# Autodesk Inventor assembly: ChassisBase
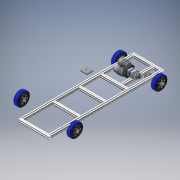
[picture p0: Inventor's stored thumbnail of the model, 180x180]
Saved by Autodesk Inventor 2018 (Build 220112000, 112)
## iProperties
Created: 2017-09-03
Part Number: ChassisBase
Document SubType Name: Assembly
Designer: snipe
Author: snipe
## Documents named in this file (12)
- E:\50000skater\Assets\ChassisBase.iam
- E:\50000skater\Assets\Resources\Profile_Len_860mm.ipt
- E:\50000skater\Assets\Resources\Profile_Len_200mm.ipt
- E:\50000skater\Assets\Resources\Profile_Len_160mm.ipt
- E:\50000skater\Assets\VPlan775dualinput.iam
- E:\50000skater\Assets\24tPulley15mm.ipt
- E:\50000skater\Assets\ShaftCollar.ipt
- E:\50000skater\Assets\PlactionWheelwithHub.iam
- E:\50000skater\Assets\PlactionWheelNoHub.iam
- E:\50000skater\Assets\THex240mm.ipt
- E:\50000skater\Assets\BearingBlock.ipt
- E:\50000skater\Assets\FlangedThunderHexBearing.ipt
## Components (21 placed, 11 different names)
1. Profile_Len_200mm:1 — Mate:1, Mate:2, Mate:3, Flush:1, Flush:2, Mate:4, Flush:3, Flush:4, Mate:10, Mate:11, Mate:13, Flush:10, Mate:23, Flush:12
2. Profile_Len_860mm:1 — Mate:3, Flush:1, Flush:2, Mate:5, Flush:5, Flush:6, Mate:7, Mate:8, Mate:9, Flush:7, Flush:8, Flush:9, Mate:30
3. Profile_Len_860mm:2 — Mate:4, Flush:3, Flush:4, Mate:16, Mate:31
4. Profile_Len_200mm:2 — Mate:5, Flush:5, Flush:6
5. Profile_Len_160mm:1 — Mate:7, Flush:9, Mate:11
6. Profile_Len_160mm:2 — Mate:8, Flush:8, Mate:10
7. Profile_Len_160mm:3 — Mate:9, Flush:7, Mate:14
8. VPlan775dualinput:1 [sub-assembly] — Flush:11, Mate:15, Mate:16, Mate:17, Mate:18, Mate:19, Mate:20, Mate:21
9. Profile_Len_200mm:3 — Mate:13, Flush:10, Mate:14, Flush:11, Mate:15
10. 24tPulley15mm:1 — Mate:17, Mate:18, Mate:19, Mate:22, Flush:13
11. ShaftCollar:1 — Mate:20, Mate:21, Mate:22
12. PlactionWheelwithHub:1 [sub-assembly] — Mate:28, Mate:29, Mate:30, Mate:35
13. PlactionWheelwithHub:2 [sub-assembly] — Mate:26, Mate:27, Mate:31, Mate:32
14. PlactionWheelNoHub:1 [sub-assembly]
15. PlactionWheelNoHub:2 [sub-assembly]
16. THex240mm:1 — Mate:23, Flush:12, Mate:24, Mate:25, Mate:26, Mate:27, Mate:28, Mate:29, Mate:33, Mate:34, Mate:36, Mate:37
17. 24tPulley15mm:2 — Mate:24, Mate:25, Flush:13
18. ShaftCollar:2 — Mate:35, Mate:36, Mate:37
19. ShaftCollar:3 — Mate:32, Mate:33, Mate:34
20. BearingBlock:1 — Mate:38, Mate:39
21. FlangedThunderHexBearing:1 — Mate:38, Mate:39
## Relationships (50: Mate 37, Flush 13)
- Mate:1: Profile_Len_200mm:1
- Mate:2: Profile_Len_200mm:1
- Mate:3: Profile_Len_200mm:1 ↔ Profile_Len_860mm:1
- Flush:1: Profile_Len_200mm:1 ↔ Profile_Len_860mm:1
- Flush:2: Profile_Len_200mm:1 ↔ Profile_Len_860mm:1
- Mate:4: Profile_Len_200mm:1 ↔ Profile_Len_860mm:2
- Flush:3: Profile_Len_200mm:1 ↔ Profile_Len_860mm:2
- Flush:4: Profile_Len_200mm:1 ↔ Profile_Len_860mm:2
- Mate:5: Profile_Len_860mm:1 ↔ Profile_Len_200mm:2
- Flush:5: Profile_Len_860mm:1 ↔ Profile_Len_200mm:2
- Flush:6: Profile_Len_860mm:1 ↔ Profile_Len_200mm:2
- Mate:7: Profile_Len_860mm:1 ↔ Profile_Len_160mm:1
- Mate:8: Profile_Len_860mm:1 ↔ Profile_Len_160mm:2
- Mate:9: Profile_Len_860mm:1 ↔ Profile_Len_160mm:3
- Flush:7: Profile_Len_860mm:1 ↔ Profile_Len_160mm:3
- Flush:8: Profile_Len_860mm:1 ↔ Profile_Len_160mm:2
- Flush:9: Profile_Len_860mm:1 ↔ Profile_Len_160mm:1
- Mate:10 (-430 mm): Profile_Len_200mm:1 ↔ Profile_Len_160mm:2
- Mate:11 (-630 mm): Profile_Len_200mm:1 ↔ Profile_Len_160mm:1
- Mate:13: Profile_Len_200mm:1 ↔ Profile_Len_200mm:3
- Flush:10: Profile_Len_200mm:1 ↔ Profile_Len_200mm:3
- Mate:14: Profile_Len_160mm:3 ↔ Profile_Len_200mm:3
- Flush:11: VPlan775dualinput:1 ↔ Profile_Len_200mm:3
- Mate:15: VPlan775dualinput:1 ↔ Profile_Len_200mm:3
- Mate:16: Profile_Len_860mm:2 ↔ VPlan775dualinput:1
- Mate:17: VPlan775dualinput:1 ↔ 24tPulley15mm:1
- Mate:18: VPlan775dualinput:1 ↔ 24tPulley15mm:1
- Mate:19: VPlan775dualinput:1 ↔ 24tPulley15mm:1
- Mate:20: VPlan775dualinput:1 ↔ ShaftCollar:1
- Mate:21: VPlan775dualinput:1 ↔ ShaftCollar:1
- Mate:22: 24tPulley15mm:1 ↔ ShaftCollar:1
- Mate:23: Profile_Len_200mm:1 ↔ THex240mm:1
- Flush:12 (-70 mm): Profile_Len_200mm:1 ↔ THex240mm:1
- Mate:24: THex240mm:1 ↔ 24tPulley15mm:2
- Mate:25: THex240mm:1 ↔ 24tPulley15mm:2
- Flush:13: 24tPulley15mm:1 ↔ 24tPulley15mm:2
- Mate:26: PlactionWheelwithHub:2 ↔ THex240mm:1
- Mate:27: PlactionWheelwithHub:2 ↔ THex240mm:1
- Mate:28: PlactionWheelwithHub:1 ↔ THex240mm:1
- Mate:29: PlactionWheelwithHub:1 ↔ THex240mm:1
- Mate:30 (10 mm): Profile_Len_860mm:1 ↔ PlactionWheelwithHub:1
- Mate:31 (10 mm): Profile_Len_860mm:2 ↔ PlactionWheelwithHub:2
- Mate:32: PlactionWheelwithHub:2 ↔ ShaftCollar:3
- Mate:33: THex240mm:1 ↔ ShaftCollar:3
- Mate:34: THex240mm:1 ↔ ShaftCollar:3
- Mate:35: PlactionWheelwithHub:1 ↔ ShaftCollar:2
- Mate:36: THex240mm:1 ↔ ShaftCollar:2
- Mate:37: THex240mm:1 ↔ ShaftCollar:2
- Mate:38: BearingBlock:1 ↔ FlangedThunderHexBearing:1
- Mate:39: BearingBlock:1 ↔ FlangedThunderHexBearing:1
